# Autodesk Inventor assembly: top
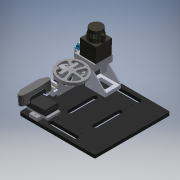
[picture p0: Inventor's stored thumbnail of the model, 180x180]
Saved by Autodesk Inventor 2017 (Build 210142000, 142)
## iProperties
Created: 2017-03-20
Part Number: top
Document SubType Name: Assembly
Designer: Naga
Author: Naga
## Documents named in this file (12)
- E:\GDrive\IEEE CS\SoutheastCon2017\Cad\top.iam
- E:\GDrive\IEEE CS\SoutheastCon2017\Cad\Chassis\TopPlateV1.ipt
- E:\GDrive\IEEE CS\SoutheastCon2017\Cad\tilt\TiltMount.iam
- E:\GDrive\IEEE CS\SoutheastCon2017\Cad\Electronics\LidarTilt.iam
- E:\GDrive\IEEE CS\SoutheastCon2017\Cad\Electronics\camera\camMounted.iam
- E:\GDrive\IEEE CS\SoutheastCon2017\Cad\Components\probe ring.ipt
- E:\GDrive\IEEE CS\SoutheastCon2017\Cad\Electronics\SS_01GL_E.iam
- E:\GDrive\IEEE CS\SoutheastCon2017\Cad\Components\limitSwitchMount.ipt
- E:\GDrive\IEEE CS\SoutheastCon2017\Cad\tilt\step\stage1Mount.iam
- E:\GDrive\IEEE CS\SoutheastCon2017\Cad\Components\probeTilit.ipt
- E:\GDrive\IEEE CS\SoutheastCon2017\Cad\tilt\TiltMountExShort.iam
- E:\GDrive\IEEE CS\SoutheastCon2017\Cad\Motors\Servo 9G.ipt
## Components (13 placed, 11 different names)
1. TopPlateV1:1 — Mate:1, Mate:3, Mate:4, Mate:6, Mate:7, Mate:8, Flush:1, Mate:11, Mate:29, Mate:31, Mate:33, Mate:35, Mate:36, Mate:47, Mate:48, Mate:53, Mate:54, Mate:55, Mate:57, Flush:61, Flush:62
2. TiltMount:1 [sub-assembly] — Mate:4, Mate:9, Mate:10, Flush:1, Mate:11
3. LidarTilt:1 [sub-assembly] — Mate:9, Mate:10, Flush:2, Flush:11, Mate:58, Mate:59, Mate:60
4. camMounted:1 [sub-assembly] — Mate:1, Mate:3, Mate:35
5. probe ring:1 — Mate:53, Mate:54, Mate:55
6. SS_01GL_E:1 [sub-assembly] — Flush:14, Mate:28, Flush:15
7. limitSwitchMount:1 — Flush:14, Mate:28, Flush:15, Mate:29, Mate:31, Mate:47
8. limitSwitchMount:2 — Mate:33, Mate:36, Mate:38, Flush:16, Mate:48
9. SS_01GL_E:2 [sub-assembly] — Mate:38, Flush:16
10. TiltMountExShort:1 [sub-assembly] — Mate:57, Flush:61, Flush:62
11. stage1Mount:1 [sub-assembly] — Mate:56, Flush:20, Flush:60
12. probeTilit:1 — Mate:56, Flush:20, Flush:60
13. Servo 9G:1 — Mate:58, Mate:59, Mate:60
## Relationships (38: Mate 28, Flush 10)
- Mate:1: TopPlateV1:1 ↔ camMounted:1
- Mate:3: TopPlateV1:1 ↔ camMounted:1
- Mate:4: TopPlateV1:1 ↔ TiltMount:1
- Mate:6: TopPlateV1:1
- Mate:7: TopPlateV1:1
- Mate:8: TopPlateV1:1
- Mate:9: TiltMount:1 ↔ LidarTilt:1
- Mate:10: TiltMount:1 ↔ LidarTilt:1
- Flush:1 (31.75 mm): TopPlateV1:1 ↔ TiltMount:1
- Mate:11: TopPlateV1:1 ↔ TiltMount:1
- Flush:2 (20.6375 mm): LidarTilt:1
- Flush:11 (22.225 mm): LidarTilt:1
- Flush:14: SS_01GL_E:1 ↔ limitSwitchMount:1
- Mate:28: SS_01GL_E:1 ↔ limitSwitchMount:1
- Flush:15 (9.0678 mm): SS_01GL_E:1 ↔ limitSwitchMount:1
- Mate:29: TopPlateV1:1 ↔ limitSwitchMount:1
- Mate:31: TopPlateV1:1 ↔ limitSwitchMount:1
- Mate:33: TopPlateV1:1 ↔ limitSwitchMount:2
- Mate:35: TopPlateV1:1 ↔ camMounted:1
- Mate:36: TopPlateV1:1 ↔ limitSwitchMount:2
- Mate:38: limitSwitchMount:2 ↔ SS_01GL_E:2
- Flush:16: limitSwitchMount:2 ↔ SS_01GL_E:2
- Mate:47: TopPlateV1:1 ↔ limitSwitchMount:1
- Mate:48: TopPlateV1:1 ↔ limitSwitchMount:2
- [Mate]: TiltMountExShort:1 ↔ stage1Mount:1
- [Mate]: TiltMountExShort:1 ↔ stage1Mount:1
- Mate:53: TopPlateV1:1 ↔ probe ring:1
- Mate:54: TopPlateV1:1 ↔ probe ring:1
- Mate:55: TopPlateV1:1 ↔ probe ring:1
- Mate:56: stage1Mount:1 ↔ probeTilit:1
- Flush:20: stage1Mount:1 ↔ probeTilit:1
- Mate:57: TopPlateV1:1 ↔ TiltMountExShort:1
- Flush:60: stage1Mount:1 ↔ probeTilit:1
- Flush:61: TopPlateV1:1 ↔ TiltMountExShort:1
- Mate:58: LidarTilt:1 ↔ Servo 9G:1
- Mate:59: LidarTilt:1 ↔ Servo 9G:1
- Mate:60: LidarTilt:1 ↔ Servo 9G:1
- Flush:62 (89.8398 mm): TopPlateV1:1 ↔ TiltMountExShort:1
